# Autodesk Inventor assembly: HeadAssembly
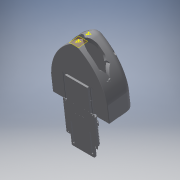
[picture p0: Inventor's stored thumbnail of the model, 180x180]
Saved by Autodesk Inventor 2018 (Build 220112000, 112)
## iProperties
Created: 2017-12-13
Part Number: HeadAssembly
Document SubType Name: Assembly
Designer: reide
Author: reide
## Documents named in this file (11)
- C:\Users\reide\OneDrive\Documents\Inventor\TSA\2018\Animatronics\Tortoise\Head\HeadAssembly.iam
- C:\Users\reide\OneDrive\Documents\Inventor\TSA\2018\Animatronics\Tortoise\Head\HeadBottom.ipt
- C:\Users\reide\OneDrive\Documents\Inventor\TSA\2018\Animatronics\Tortoise\Head\HeadTop.ipt
- C:\Users\reide\OneDrive\Documents\Inventor\TSA\2018\Animatronics\Tortoise\Head\HeadBase.iam
- C:\Users\reide\OneDrive\Documents\Inventor\TSA\2018\Animatronics\Tortoise\Syringe1mL\Syringe.iam
- C:\Users\reide\OneDrive\Documents\Inventor\TSA\2018\Animatronics\Tortoise\Head\SyringeAttachment.ipt
- C:\Users\reide\OneDrive\Documents\Inventor\TSA\2018\Animatronics\Tortoise\Head\HeadLever.ipt
- C:\Users\reide\OneDrive\Documents\Inventor\TSA\2018\Animatronics\Tortoise\Syringe1mL\SyringEnd.ipt
- C:\Users\reide\OneDrive\Documents\Inventor\TSA\2018\Animatronics\Tortoise\Head\Face.ipt
- C:\Users\reide\OneDrive\Documents\Inventor\TSA\2018\Animatronics\Tortoise\Head\FlexHinge.ipt
- C:\Users\reide\OneDrive\Documents\Inventor\TSA\2018\Animatronics\Tortoise\Head\HeadBottom1.ipt
## Components (12 placed, 10 different names)
1. HeadTop:1 — Flush:10, Flush:11, Mate:23, Mate:24, Mate:27, Mate:28, Flush:13, Flush:14
2. Syringe:2 [sub-assembly] — Mate:21
3. SyringeAttachment:4 — Mate:16, Mate:17, Mate:18
4. SyringeAttachment:5 — Mate:14, Mate:15
5. HeadBottom:2 — Mate:14, Mate:15, Mate:16, Mate:17, Mate:18, Mate:19, Mate:20, Mate:25, Mate:26, Flush:12, Flush:13, Flush:14, Flush:15, Mate:29, Mate:30
6. HeadLever:2 — Mate:19, Mate:20, Mate:22
7. SyringEnd:1 — Mate:21, Mate:22
8. Face:1 — Flush:10, Mate:27, Mate:28
9. FlexHinge:1 — Flush:11
10. FlexHinge:2 — Mate:23, Mate:24, Mate:25
11. HeadBase:2 [sub-assembly] — Mate:26, Flush:12
12. HeadBottom1:1 — Flush:15, Mate:29, Mate:30
## Relationships (28: Mate 20, Flush 8)
- [Mate] (10 mm): Syringe:2 ↔ SyringeAttachment:4
- [Mate]: Syringe:2 ↔ SyringeAttachment:4
- [Flush]: Syringe:2 ↔ SyringeAttachment:4
- [Mate]: Syringe:2 ↔ SyringeAttachment:5
- [Flush]: SyringeAttachment:4 ↔ SyringeAttachment:5
- Mate:14 (0.2 mm): SyringeAttachment:5 ↔ HeadBottom:2
- Mate:15 (0.2 mm): SyringeAttachment:5 ↔ HeadBottom:2
- Mate:16 (0.2 mm): SyringeAttachment:4 ↔ HeadBottom:2
- Mate:17 (0.2 mm): SyringeAttachment:4 ↔ HeadBottom:2
- Mate:18: SyringeAttachment:4 ↔ HeadBottom:2
- Mate:19 (0.25 mm): HeadBottom:2 ↔ HeadLever:2
- Mate:20: HeadBottom:2 ↔ HeadLever:2
- Mate:21: Syringe:2 ↔ SyringEnd:1
- Mate:22: HeadLever:2 ↔ SyringEnd:1
- Flush:10: HeadTop:1 ↔ Face:1
- Flush:11: HeadTop:1 ↔ FlexHinge:1
- Mate:23: HeadTop:1 ↔ FlexHinge:2
- Mate:24: HeadTop:1 ↔ FlexHinge:2
- Mate:25: HeadBottom:2 ↔ FlexHinge:2
- Mate:26: HeadBottom:2 ↔ HeadBase:2
- Flush:12: HeadBottom:2 ↔ HeadBase:2
- Mate:27: HeadTop:1 ↔ Face:1
- Mate:28: HeadTop:1 ↔ Face:1
- Flush:13: HeadTop:1 ↔ HeadBottom:2
- Flush:14: HeadTop:1 ↔ HeadBottom:2
- Flush:15: HeadBottom:2 ↔ HeadBottom1:1
- Mate:29: HeadBottom:2 ↔ HeadBottom1:1
- Mate:30 (0.25 mm): HeadBottom:2 ↔ HeadBottom1:1
## Named parameters: d34_d32 = 0 mm, d35_d33 = 0 mm, d36_d28 = 10 mm, d37_d29 = 0 mm, d38_d30 = 0 mm
